# Autodesk Inventor assembly: IR_Transmitter
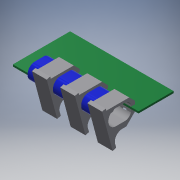
[picture p0: Inventor's stored thumbnail of the model, 180x180]
Saved by Autodesk Inventor 2018 (Build 220112000, 112)
## iProperties
Created: 2018-02-04
Part Number: IR_Transmitter
Document SubType Name: Assembly
Designer: Mandus
Author: Mandus
## Documents named in this file (4)
- C:\Users\Mandus\Dropbox\Skola\Projekt\Kretsn_Brillz_V2\3D\IR_Transmitter.iam
- C:\Users\Mandus\Dropbox\Skola\Projekt\Kretsn_Brillz_V2\3D\IR_PCB_Inventor.ipt
- C:\Users\Mandus\Dropbox\Skola\Projekt\Kretsn_Brillz_V2\3D\Powerbank.ipt
- C:\Users\Mandus\Dropbox\Skola\Projekt\Kretsn_Brillz_V2\3D\Stand_Front.ipt
## Components (5 placed, 3 different names)
1. IR_PCB_Inventor:1 — Mate:1, Mate:2, Mate:3, Flush:1, Mate:4, Mate:5, Mate:6, Mate:7
2. Powerbank:1 — Mate:1, Mate:2, Mate:3
3. Stand_Front:1 — Flush:1
4. Stand_Front:2 — Mate:4, Mate:6
5. Stand_Front:3 — Mate:5, Mate:7
## Relationships (8: Mate 7, Flush 1)
- Mate:1: IR_PCB_Inventor:1 ↔ Powerbank:1
- Mate:2: IR_PCB_Inventor:1 ↔ Powerbank:1
- Mate:3: IR_PCB_Inventor:1 ↔ Powerbank:1
- Flush:1: IR_PCB_Inventor:1 ↔ Stand_Front:1
- Mate:4: IR_PCB_Inventor:1 ↔ Stand_Front:2
- Mate:5: IR_PCB_Inventor:1 ↔ Stand_Front:3
- Mate:6: IR_PCB_Inventor:1 ↔ Stand_Front:2
- Mate:7: IR_PCB_Inventor:1 ↔ Stand_Front:3
